# Autodesk Inventor assembly: Side Panel
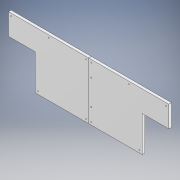
[picture p0: Inventor's stored thumbnail of the model, 180x180]
Saved by Autodesk Inventor 2017 SP1 (Build 210196100, 196)
## iProperties
Created: 2017-08-09
Part Number: Side Panel
Document SubType Name: Assembly
Designer: Zach
Author: Zach
## Documents named in this file (3)
- C:\Users\Zach\Documents\GitHub\tr1\src\Base\Side Panel\Side Panel.iam
- C:\Users\Zach\Documents\GitHub\tr1\src\Base\Side Panel\SP003b.ipt
- C:\Users\Zach\Documents\GitHub\tr1\src\Base\Side Panel\SP004b.ipt
## Components (2 placed, 2 different names)
1. SP003b:1 — Mate:1, Mate:2, Mate:3
2. SP004b:1 — Mate:1, Mate:2, Mate:3
## Relationships (3: Mate 3)
- Mate:1: SP003b:1 ↔ SP004b:1
- Mate:2: SP003b:1 ↔ SP004b:1
- Mate:3: SP003b:1 ↔ SP004b:1
